# Autodesk Inventor assembly: LAMP_OUTDOOR_BATTERY
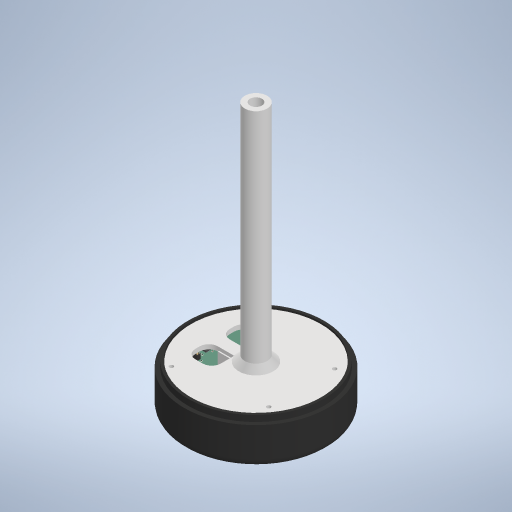
[picture p0: Inventor's stored thumbnail of the model, 512x512]
Saved by Autodesk Inventor 2024 (Build 280153000, 153)
## iProperties
Created: 2025-01-19
Part Number: LAMP_OUTDOOR_BATTERY
Document SubType Name: Assembly
Designer: malam
Author: malam
## Documents named in this file (7)
- C:\Users\malam\Documents\6 - PROJET\15 - LAMP OUTDOOR BATTERY\LAMP-OUTDOOR-BATTERY\2 - CONCEPTION 3D\20 - CONCEPTION 3D\LAMP_OUTDOOR_BATTERY.iam
- C:\Users\malam\Documents\6 - PROJET\15 - LAMP OUTDOOR BATTERY\LAMP-OUTDOOR-BATTERY\2 - CONCEPTION 3D\20 - CONCEPTION 3D\Socle test mesure.ipt
- C:\Users\malam\Documents\6 - PROJET\15 - LAMP OUTDOOR BATTERY\LAMP-OUTDOOR-BATTERY\2 - CONCEPTION 3D\20 - CONCEPTION 3D\18650Battery.ipt
- C:\Users\malam\Documents\6 - PROJET\15 - LAMP OUTDOOR BATTERY\LAMP-OUTDOOR-BATTERY\2 - CONCEPTION 3D\20 - CONCEPTION 3D\Bocal.ipt
- C:\Users\malam\Documents\6 - PROJET\15 - LAMP OUTDOOR BATTERY\LAMP-OUTDOOR-BATTERY\2 - CONCEPTION 3D\20 - CONCEPTION 3D\Lamp_PCB.iam
- C:\Users\malam\Documents\6 - PROJET\15 - LAMP OUTDOOR BATTERY\LAMP-OUTDOOR-BATTERY\2 - CONCEPTION 3D\20 - CONCEPTION 3D\Switch_On_Off.ipt
- C:\Users\malam\Documents\6 - PROJET\15 - LAMP OUTDOOR BATTERY\LAMP-OUTDOOR-BATTERY\2 - CONCEPTION 3D\20 - CONCEPTION 3D\Support_led.ipt
## Components (7 placed, 6 different names)
1. 18650Battery:2 — Affleurement:1, Placage:19, Affleurement:2
2. 18650Battery:3 — Affleurement:1, Placage:20, Placage:25
3. Bocal:1 — Placage:26, Placage:27
4. Lamp_PCB:1 [sub-assembly] — Placage:16, Placage:17, Placage:18
5. Switch_On_Off:1 — Placage:21, Placage:22, Placage:23
6. Support_led:1 — Placage:24, Placage:25
7. Socle test mesure:1 — Placage:16, Placage:17, Placage:18, Placage:19, Placage:20, Affleurement:2, Placage:21, Placage:22, Placage:23, Placage:24, Placage:26, Placage:27
## Relationships (14: Mate 12, Flush 2)
- Affleurement:1 [Flush]: 18650Battery:2 ↔ 18650Battery:3
- Placage:16 [Mate]: Lamp_PCB:1 ↔ Socle test mesure:1
- Placage:17 [Mate]: Lamp_PCB:1 ↔ Socle test mesure:1
- Placage:18 [Mate] (0.2 mm): Lamp_PCB:1 ↔ Socle test mesure:1
- Placage:19 [Mate]: 18650Battery:2 ↔ Socle test mesure:1
- Placage:20 [Mate]: 18650Battery:3 ↔ Socle test mesure:1
- Affleurement:2 [Flush] (-5.5 mm): 18650Battery:2 ↔ Socle test mesure:1
- Placage:21 [Mate] (0.15 mm): Switch_On_Off:1 ↔ Socle test mesure:1
- Placage:22 [Mate] (0.25 mm): Switch_On_Off:1 ↔ Socle test mesure:1
- Placage:23 [Mate]: Switch_On_Off:1 ↔ Socle test mesure:1
- Placage:24 [Mate]: Support_led:1 ↔ Socle test mesure:1
- Placage:25 [Mate]: 18650Battery:3 ↔ Support_led:1
- Placage:26 [Mate]: Bocal:1 ↔ Socle test mesure:1
- Placage:27 [Mate]: Bocal:1 ↔ Socle test mesure:1
